# Autodesk Inventor assembly: Swing_Arm
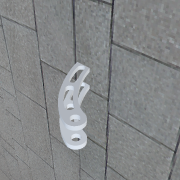
[picture p0: Inventor's stored thumbnail of the model, 180x180]
Saved by Autodesk Inventor 2016 (Build 200138000, 138)
## iProperties
Created: 2015-05-19
Part Number: Swing_Arm
Document SubType Name: Assembly
Designer: Yann
Author: Yann
## Documents named in this file (5)
- C:\Users\Yann\Documents\GitHub\BIKAIR_CAD\Source\Rear_Train\Swing_Arm.iam
- C:\Users\Yann\Documents\GitHub\BIKAIR_CAD\Source\Rear_Train\Profile.ipt
- C:\Users\Yann\Documents\GitHub\BIKAIR_CAD\Source\Rear_Train\Profile_MIR.ipt
- C:\Users\Yann\Documents\GitHub\BIKAIR_CAD\Source\Rear_Train\Profile_Straight.ipt
- C:\Users\Yann\Documents\GitHub\BIKAIR_CAD\Source\Rear_Train\Profile_Straight_MIR.ipt
## Components (4 placed, 4 different names)
1. Profile_MIR:1 — Mate:2, Mate:3
2. Profile:1 — Mate:1, Flush:1, Mate:2
3. Profile_Straight:1 — Mate:4, Mate:5
4. Profile_Straight_MIR:1 — Flush:2, Mate:6
## Relationships (8: Mate 6, Flush 2)
- Mate:1: Profile:1
- Flush:1 (55 mm): Profile:1
- Mate:2: Profile_MIR:1 ↔ Profile:1
- Mate:3: Profile_MIR:1
- Mate:4: Profile_Straight:1
- Mate:5 (55 mm): Profile_Straight:1
- Flush:2 (-55 mm): Profile_Straight_MIR:1
- Mate:6: Profile_Straight_MIR:1
